# Autodesk Inventor assembly: throwerAssembly
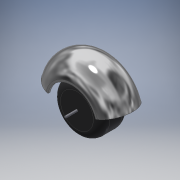
[picture p0: Inventor's stored thumbnail of the model, 180x180]
Saved by Autodesk Inventor 2016 (Build 200138000, 138)
## iProperties
Created: 2015-11-01
Part Number: throwerAssembly
Document SubType Name: Assembly
Designer: rossmosier
Author: rossmosier
## Documents named in this file (4)
- C:\Users\rossmosier\Documents\CAD Team\CADTeam\Thrower\throwerAssembly.iam
- C:\Users\rossmosier\Documents\CAD Team\CADTeam\Thrower\flyWheel.ipt
- C:\Users\rossmosier\Documents\CAD Team\CADTeam\Thrower\throwerAssembly\Design Accelerator\Shaft1.iam
- C:\Users\rossmosier\Documents\CAD Team\CADTeam\Thrower\throwerRamp.ipt
## Components (3 placed, 3 different names)
1. flyWheel:1 — Rotational:1
2. Shaft:1 [sub-assembly] — Rotational:1
3. throwerRamp:1
## Relationships (1: RevoluteJoint 1)
- Rotational:1 [RevoluteJoint] (-12.7 mm): flyWheel:1 ↔ Shaft:1
